# Autodesk Inventor assembly: Dedo con plataforma
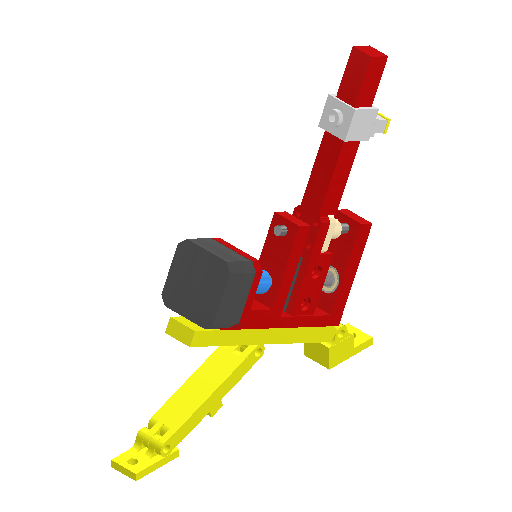
[picture p0: Inventor's stored thumbnail of the model, 512x512]
Saved by Autodesk Inventor 2024 (Build 280153000, 153)
## iProperties
Created: 2023-05-25
Part Number: Dedo con plataforma
Document SubType Name: Assembly
Designer: ferna
Author: ferna
## Documents named in this file (3)
- C:\Users\ferna\OneDrive - Universidad Católica de Chile\Bocas\RobotFlautista\Dedo con plataforma.iam
- C:\Users\ferna\OneDrive - Universidad Católica de Chile\Bocas\NuevosDedos\Dedo - 1.iam
- C:\Users\ferna\OneDrive - Universidad Católica de Chile\Bocas\NuevosDedos\Lifter 1.iam
## Components (2 placed, 2 different names)
1. Dedo - 1:1 [sub-assembly] — Mate:1, Flush:1, Flush:2
2. Lifter 1:1 [sub-assembly] — Mate:1, Flush:1, Flush:2
## Relationships (3: Flush 2, Mate 1)
- Mate:1: Dedo - 1:1 ↔ Lifter 1:1
- Flush:1: Dedo - 1:1 ↔ Lifter 1:1
- Flush:2: Dedo - 1:1 ↔ Lifter 1:1
